# Autodesk Inventor assembly: Short Roller Assembly
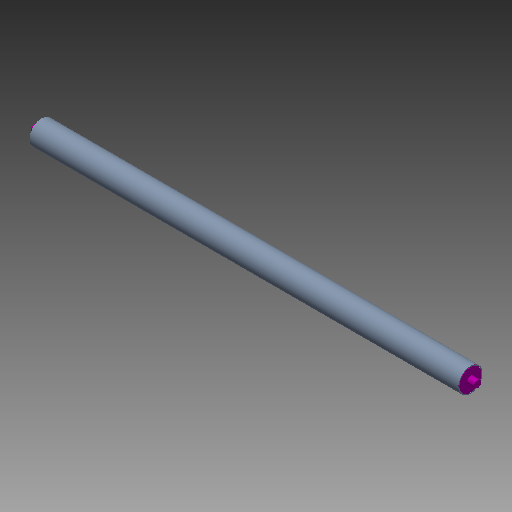
[picture p0: Inventor's stored thumbnail of the model, 512x512]
Saved by Autodesk Inventor 2017 (Build 210142000, 142)
## iProperties
Created: 2017-01-14
Part Number: Short Roller Assembly
Document SubType Name: Assembly
Designer: Ben
Author: Ben
## Documents named in this file (3)
- C:\Users\Ben\Desktop\Projects\2017 Robot\Ball Intake\Short Roller Assembly.iam
- C:\Users\Ben\Desktop\Projects\2017 Robot\Ball Intake\1in Short PVC Roller.ipt
- C:\Users\Ben\Desktop\Projects\2017 Robot\Ball Intake\1in PVC End Cap.ipt
## Components (3 placed, 2 different names)
1. 1in Short PVC Roller:1 — Insert:3, Insert:4
2. 1in PVC End Cap:1 — Insert:3
3. 1in PVC End Cap:2 — Insert:4
## Relationships (2: Insert 2)
- Insert:3: 1in Short PVC Roller:1 ↔ 1in PVC End Cap:1
- Insert:4: 1in Short PVC Roller:1 ↔ 1in PVC End Cap:2
